# Autodesk Inventor assembly: intake_gearbox_outer_mirrored
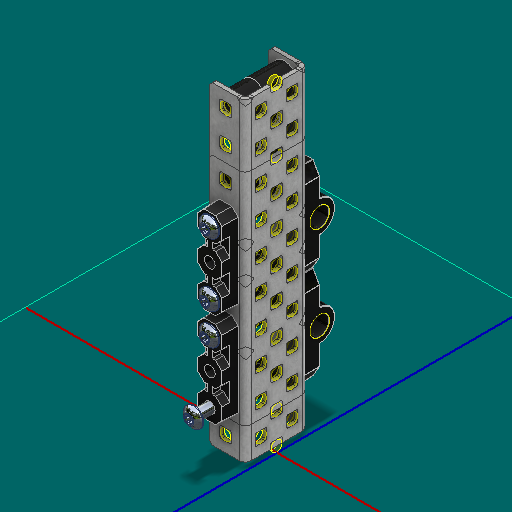
[picture p0: Inventor's stored thumbnail of the model, 512x512]
Saved by Autodesk Inventor 2025 (Build 290162000, 162)
## iProperties
Created: 2024-08-19
Part Number: intake_gearbox_outer_mirrored
Document SubType Name: Assembly
Designer: averey
Author: averey
## Documents named in this file (14)
- C:\Users\avere\vex_robotics_high_stakes\hardware\cad\ATLAS\tower\structure\structure_half_mirrored\intake_gearbox_outer_mirrored.iam
- C:\Users\avere\vex_robotics_high_stakes\hardware\cad\ATLAS\tower\structure\structure_half_mirrored\Alu C 1x2x1x8_mirrored.ipt
- C:\Users\avere\vex_robotics_high_stakes\hardware\cad\ATLAS\tower\structure\structure_half_mirrored\HS Pillow Bearing Block_mirrored.ipt
- C:\Users\avere\vex_robotics_high_stakes\hardware\cad\VEX-CAD-Inventor\Motion\Spacers\Spacer Nylon .375 OD\NSpacer .375 OD x .375.ipt
- C:\Users\avere\vex_robotics_high_stakes\hardware\cad\VEX-CAD-Inventor\Motion\Spacers\Spacer Nylon .375 OD.ipt
- C:\Users\avere\vex_robotics_high_stakes\hardware\cad\VEX-CAD-Inventor\Motion\Spacers\Spacer Nylon .375 OD\NSpacer .375 OD x .500.ipt
- C:\Users\avere\vex_robotics_high_stakes\hardware\cad\ATLAS\tower\structure\structure_half_mirrored\Bearing Flat_mirrored.ipt
- C:\Users\avere\vex_robotics_high_stakes\hardware\cad\VEX-CAD-Inventor\Structure\Hardware\Screw Steel - Star\SScrew Star Smooth 1.500.ipt
- C:\Users\avere\vex_robotics_high_stakes\hardware\cad\VEX-CAD-Inventor\Structure\Hardware\Screw Steel - Star.ipt
- C:\Users\avere\vex_robotics_high_stakes\hardware\cad\ATLAS\tower\structure\structure_half_mirrored\Nut Thin Nylock_mirrored.ipt
- C:\Users\avere\vex_robotics_high_stakes\hardware\cad\ATLAS\tower\structure\structure_half_mirrored\Alu C 1x2x1x10_mirrored.ipt
- C:\Users\avere\vex_robotics_high_stakes\hardware\cad\ATLAS\tower\structure\structure_half_mirrored\HS Bearing Flat_mirrored.ipt
- C:\Users\avere\vex_robotics_high_stakes\hardware\cad\ATLAS\tower\structure\structure_half_mirrored\Alu C 1x2x1x9_mirrored.ipt
- C:\Users\avere\vex_robotics_high_stakes\hardware\cad\VEX-CAD-Inventor\Structure\Hardware\Screw Steel - Star\SScrew Star Smooth 1.750.ipt
## Components (28 placed, 11 different names)
1. Alu C 1x2x1x8_mirrored:1 — Insert:33, Mate:5, Mate:4, Insert:32, Mate:6, Insert:34
2. HS Pillow Bearing Block_mirrored:1 — Insert:18, Insert:20, Insert:12, Insert:11
3. NSpacer .375 OD x .375:1 — Insert:18, Insert:7
4. NSpacer .375 OD x .500:2 — Insert:33, Insert:7, Insert:17
5. NSpacer .375 OD x .375:3 — Insert:20, Insert:8
6. NSpacer .375 OD x .500:4 — Mate:5, Insert:8, Insert:19
7. Bearing Flat_mirrored:1 — Insert:19, Insert:17, Insert:10, Insert:9
8. SScrew Star Smooth 1.500:1 — Insert:10
9. SScrew Star Smooth 1.500:2 — Insert:9
10. Nut Thin Nylock_mirrored:1 — Insert:12
11. Nut Thin Nylock_mirrored:2 — Insert:11
12. HS Pillow Bearing Block_mirrored:2 — Insert:29, Insert:27, Insert:26, Mate:6
13. NSpacer .375 OD x .375:5 — Insert:29, Insert:40, Insert:30
14. NSpacer .375 OD x .500:6 — Mate:4, Insert:30
15. NSpacer .375 OD x .375:7 — Insert:23
16. NSpacer .375 OD x .500:8 — Insert:32, Insert:23, Insert:30
17. Bearing Flat_mirrored:2 — Insert:30, Insert:24, Mate:8, Insert:41
18. SScrew Star Smooth 1.500:3 — Insert:24
19. Nut Thin Nylock_mirrored:3 — Insert:27
20. Nut Thin Nylock_mirrored:4 — Insert:26
21. Alu C 1x2x1x10_mirrored:1 — Mate:6, Insert:34, Mate:7, Insert:35, Insert:39, Insert:38
22. HS Bearing Flat_mirrored:1 — Mate:7, Insert:35
23. NSpacer .375 OD x .375:9 — Insert:36
24. NSpacer .375 OD x .500:10 — Insert:39, Insert:36
25. NSpacer .375 OD x .375:11 — Insert:37
26. NSpacer .375 OD x .500:12 — Insert:38, Insert:37
27. Alu C 1x2x1x9_mirrored:1 — Mate:8, Insert:40, Mate:6
28. SScrew Star Smooth 1.750:4 — Insert:41
## Relationships (33: Insert 27, Mate 6)
- Insert:18 (1.5875 mm): HS Pillow Bearing Block_mirrored:1 ↔ NSpacer .375 OD x .375:1
- Insert:33: Alu C 1x2x1x8_mirrored:1 ↔ NSpacer .375 OD x .500:2
- Insert:7: NSpacer .375 OD x .375:1 ↔ NSpacer .375 OD x .500:2
- Insert:20 (1.5875 mm): HS Pillow Bearing Block_mirrored:1 ↔ NSpacer .375 OD x .375:3
- Mate:5: Alu C 1x2x1x8_mirrored:1 ↔ NSpacer .375 OD x .500:4
- Insert:8: NSpacer .375 OD x .375:3 ↔ NSpacer .375 OD x .500:4
- Insert:19 (1.5875 mm): NSpacer .375 OD x .500:4 ↔ Bearing Flat_mirrored:1
- Insert:17 (1.5875 mm): NSpacer .375 OD x .500:2 ↔ Bearing Flat_mirrored:1
- Insert:10: Bearing Flat_mirrored:1 ↔ SScrew Star Smooth 1.500:1
- Insert:9: Bearing Flat_mirrored:1 ↔ SScrew Star Smooth 1.500:2
- Insert:12: HS Pillow Bearing Block_mirrored:1 ↔ Nut Thin Nylock_mirrored:1
- Insert:11: HS Pillow Bearing Block_mirrored:1 ↔ Nut Thin Nylock_mirrored:2
- Insert:29 (1.5875 mm): HS Pillow Bearing Block_mirrored:2 ↔ NSpacer .375 OD x .375:5
- Mate:4: Alu C 1x2x1x8_mirrored:1 ↔ NSpacer .375 OD x .500:6
- Insert:32: Alu C 1x2x1x8_mirrored:1 ↔ NSpacer .375 OD x .500:8
- Insert:23: NSpacer .375 OD x .375:7 ↔ NSpacer .375 OD x .500:8
- Insert:30 (1.5875 mm): NSpacer .375 OD x .500:8 ↔ Bearing Flat_mirrored:2
- Insert:24: Bearing Flat_mirrored:2 ↔ SScrew Star Smooth 1.500:3
- Insert:27: HS Pillow Bearing Block_mirrored:2 ↔ Nut Thin Nylock_mirrored:3
- Insert:26: HS Pillow Bearing Block_mirrored:2 ↔ Nut Thin Nylock_mirrored:4
- Mate:6: Alu C 1x2x1x8_mirrored:1 ↔ Alu C 1x2x1x10_mirrored:1
- Insert:34: Alu C 1x2x1x8_mirrored:1 ↔ Alu C 1x2x1x10_mirrored:1
- Mate:7: Alu C 1x2x1x10_mirrored:1 ↔ HS Bearing Flat_mirrored:1
- Insert:35: Alu C 1x2x1x10_mirrored:1 ↔ HS Bearing Flat_mirrored:1
- Insert:39: Alu C 1x2x1x10_mirrored:1 ↔ NSpacer .375 OD x .500:10
- Insert:36: NSpacer .375 OD x .375:9 ↔ NSpacer .375 OD x .500:10
- Insert:38: Alu C 1x2x1x10_mirrored:1 ↔ NSpacer .375 OD x .500:12
- Insert:37: NSpacer .375 OD x .375:11 ↔ NSpacer .375 OD x .500:12
- Mate:8: Bearing Flat_mirrored:2 ↔ Alu C 1x2x1x9_mirrored:1
- Insert:40: NSpacer .375 OD x .375:5 ↔ Alu C 1x2x1x9_mirrored:1
- Insert:41 (6.35 mm): Bearing Flat_mirrored:2 ↔ SScrew Star Smooth 1.750:4
- Insert:30: NSpacer .375 OD x .375:5 ↔ NSpacer .375 OD x .500:6
- Mate:6: HS Pillow Bearing Block_mirrored:2 ↔ Alu C 1x2x1x9_mirrored:1
